# Autodesk Inventor assembly: 1_Base
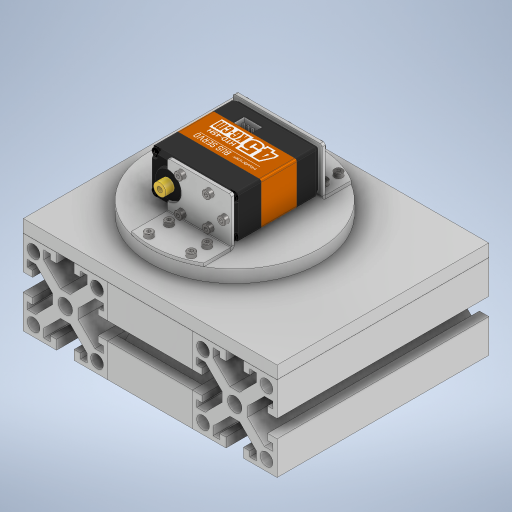
[picture p0: Inventor's stored thumbnail of the model, 512x512]
Saved by Autodesk Inventor 2024.1 (Build 281209000, 209)
## iProperties
Created: 2023-08-24
Part Number: 1_Base
Document SubType Name: Assembly
Designer: chanh
Author: chanh
## Documents named in this file (19)
- C:\Users\chanh\OneDrive - 연세대학교 (Yonsei University)\로봇\Humanoid\Roboin Humanoid Project\Inventor\rh_plus_7_axis_robot_arm_hardware\Assembly\2_Arm.iam
- C:\Users\chanh\OneDrive - 연세대학교 (Yonsei University)\로봇\Humanoid\Roboin Humanoid Project\Inventor\rh_plus_7_axis_robot_arm_hardware\Part\HTD-45H, Horn\HTD-45H\HTD-45H.ipt
- C:\Users\chanh\OneDrive - 연세대학교 (Yonsei University)\로봇\Humanoid\Roboin Humanoid Project\Inventor\rh_plus_7_axis_robot_arm_hardware\Part\Frame\axis_1_top_frame.ipt
- C:\Users\chanh\OneDrive - 연세대학교 (Yonsei University)\로봇\Humanoid\Roboin Humanoid Project\Inventor\rh_plus_7_axis_robot_arm_hardware\Part\Other Parts\Aluminum_Profile_4040_100.14mm_top.ipt
- C:\Users\chanh\OneDrive - 연세대학교 (Yonsei University)\로봇\Humanoid\Roboin Humanoid Project\Inventor\rh_plus_7_axis_robot_arm_hardware\Part\Other Parts\Aluminum_Profile_4040_40.10mm_right.ipt
- C:\Users\chanh\OneDrive - 연세대학교 (Yonsei University)\로봇\Humanoid\Roboin Humanoid Project\Inventor\rh_plus_7_axis_robot_arm_hardware\Part\Other Parts\Aluminum_Profile_4040_40.10mm_left.ipt
- C:\Users\chanh\OneDrive - 연세대학교 (Yonsei University)\로봇\Humanoid\Roboin Humanoid Project\Inventor\rh_plus_7_axis_robot_arm_hardware\Part\Other Parts\Aluminum_Profile_4040_100.14mm_bottom.ipt
- C:\Users\chanh\OneDrive - 연세대학교 (Yonsei University)\로봇\Humanoid\Roboin Humanoid Project\Inventor\rh_plus_7_axis_robot_arm_hardware\Part\HTD-45H, Horn\HTD-45H\M2x32.ipt
- C:\Users\chanh\OneDrive - 연세대학교 (Yonsei University)\로봇\Humanoid\Roboin Humanoid Project\Inventor\rh_plus_7_axis_robot_arm_hardware\Part\HTD-45H, Horn\Horn\Top Horn.ipt
- C:\Users\chanh\OneDrive - 연세대학교 (Yonsei University)\로봇\Humanoid\Roboin Humanoid Project\Inventor\rh_plus_7_axis_robot_arm_hardware\Part\Bolt, Bearing\M2x6 Round Bolt.ipt
- C:\Users\chanh\OneDrive - 연세대학교 (Yonsei University)\로봇\Humanoid\Roboin Humanoid Project\Inventor\rh_plus_7_axis_robot_arm_hardware\Part\Bolt, Bearing\M2x35 Round Bolt.ipt
- C:\Users\chanh\OneDrive - 연세대학교 (Yonsei University)\로봇\Humanoid\Roboin Humanoid Project\Inventor\rh_plus_7_axis_robot_arm_hardware\Part\Frame\axis_2_bottom_frame.ipt
- C:\Users\chanh\OneDrive - 연세대학교 (Yonsei University)\로봇\Humanoid\Roboin Humanoid Project\Inventor\rh_plus_7_axis_robot_arm_hardware\Part\Bolt, Bearing\AXK5070+AS Bearing.ipt
- C:\Users\chanh\OneDrive - 연세대학교 (Yonsei University)\로봇\Humanoid\Roboin Humanoid Project\Inventor\rh_plus_7_axis_robot_arm_hardware\Part\Bolt, Bearing\M2x6 Bolt.ipt
- C:\Users\chanh\OneDrive - 연세대학교 (Yonsei University)\로봇\Humanoid\Roboin Humanoid Project\Inventor\rh_plus_7_axis_robot_arm_hardware\Part\HTD-45H, Horn\HTD-45H\HTD-45H.iam
- C:\Users\chanh\OneDrive - 연세대학교 (Yonsei University)\로봇\Humanoid\Roboin Humanoid Project\Inventor\rh_plus_7_axis_robot_arm_hardware\Part\HTD-45H, Horn\Horn\M3x6.ipt
- C:\Users\chanh\OneDrive - 연세대학교 (Yonsei University)\로봇\Humanoid\Roboin Humanoid Project\Inventor\rh_plus_7_axis_robot_arm_hardware\Part\Frame\axis_2_bottom_L_frame(top).ipt
- C:\Users\chanh\OneDrive - 연세대학교 (Yonsei University)\로봇\Humanoid\Roboin Humanoid Project\Inventor\rh_plus_7_axis_robot_arm_hardware\Part\Frame\axis_2_bottom_L_frame(bottom).ipt
- C:\Users\chanh\OneDrive - 연세대학교 (Yonsei University)\로봇\Humanoid\Roboin Humanoid Project\Inventor\rh_plus_7_axis_robot_arm_hardware\Part\Bolt, Bearing\M2x4 Bolt.ipt
## Components (47 placed, 17 different names)
1. M2x4 Bolt:1 — Rigid:23
2. M2x4 Bolt:2 — Rigid:24
3. M2x4 Bolt:3 — Rigid:25
4. M2x4 Bolt:4 — Rigid:26
5. M2x4 Bolt:5 — Rigid:27
6. M2x4 Bolt:6 — Rigid:28
7. M2x4 Bolt:7 — Rigid:29
8. M2x4 Bolt:8 — Rigid:30
9. M2x4 Bolt:9 — Rigid:31
10. M2x4 Bolt:10 — Rigid:32
11. M2x4 Bolt:11 — Rigid:33
12. M2x4 Bolt:12 — Rigid:34
13. M2x4 Bolt:13 — Rigid:38
14. M2x4 Bolt:14 — Rigid:39
15. M2x4 Bolt:15 — Rigid:41
16. M2x4 Bolt:16 — Rigid:37
17. M2x4 Bolt:17 — Rigid:35
18. M2x4 Bolt:18 — Rigid:36
19. M2x4 Bolt:19 — Rigid:40
20. M2x4 Bolt:20 — Rigid:42
21. M2x4 Bolt:21 — Rigid:43
22. Aluminum_Profile_4040_100.14mm_top:1 — Flush:13, Flush:14, Mate:2, Mate:3, Flush:15, Flush:16, Mate:4, Flush:17, Flush:18, Mate:6
23. Aluminum_Profile_4040_40.10mm_right:1 — Mate:3, Flush:15, Flush:16
24. Aluminum_Profile_4040_40.10mm_left:1 — Mate:4, Flush:17, Flush:18, Mate:5, Flush:20
25. Aluminum_Profile_4040_100.14mm_bottom:1 — Flush:19, Mate:5, Flush:20
26. HTD-45H:1 — Mate:1, Flush:1, Flush:2, Flush:12, Flush:13, Flush:14, Mate:2, Flush:19, Rigid:1, Rigid:2, Rotational:1, Mate:7, Mate:8
27. axis_1_top_frame:1 — Flush:11, Flush:12, Mate:6, Rigid:11, Rigid:12, Rigid:13, Rigid:14, Rigid:15, Rigid:16, Rigid:17, Mate:9
28. HTD-45H:2 [sub-assembly] — Flush:21, Mate:11, Flush:23, Flush:24, Mate:13, Mate:17
29. axis_2_bottom_frame:1 — Rigid:10, Rigid:18, Rigid:19, Rigid:20, Rigid:21, Flush:21, Mate:11, Mate:14
30. axis_2_bottom_L_frame(top):1 — Flush:23, Flush:24, Mate:13, Mate:14, Rigid:23, Rigid:24, Rigid:25, Rigid:26, Rigid:27, Rigid:28, Rigid:29, Rigid:30, Rigid:31
31. axis_2_bottom_L_frame(bottom):1 — Mate:17, Rigid:32, Rigid:33, Rigid:34, Rigid:35, Rigid:36, Rigid:37, Rigid:38, Rigid:39, Rigid:40, Rigid:41, Rigid:42, Rigid:43
32. M2x32:1 — Rigid:2
33. M2x32:2 — Rigid:1
34. Top Horn:1 — Rotational:1, Rigid:10, Rigid:22
35. M3x6:1 — Rigid:22
36. M2x6 Round Bolt:3 — Rigid:16
37. M2x6 Round Bolt:4 — Rigid:17
38. M2x6 Round Bolt:5 — Rigid:15
39. AXK5070+AS Bearing:1 — Mate:7, Mate:8, Mate:9
40. M2x6 Round Bolt:1 — Rigid:14
41. M2x6 Round Bolt:2 — Rigid:13
42. M2x35 Round Bolt:1 — Rigid:11
43. M2x35 Round Bolt:2 — Rigid:12
44. M2x6 Bolt:1 — Rigid:18
45. M2x6 Bolt:2 — Rigid:19
46. M2x6 Bolt:3 — Rigid:20
47. M2x6 Bolt:4 — Rigid:21
## Relationships (65: WeldJoint 36, Flush 15, Mate 13, RevoluteJoint 1)
- Mate:1: HTD-45H:1
- Flush:1: HTD-45H:1
- Flush:2: HTD-45H:1
- Flush:11: axis_1_top_frame:1
- Flush:12: HTD-45H:1 ↔ axis_1_top_frame:1
- Flush:13: Aluminum_Profile_4040_100.14mm_top:1 ↔ HTD-45H:1
- Flush:14: Aluminum_Profile_4040_100.14mm_top:1 ↔ HTD-45H:1
- Mate:2: Aluminum_Profile_4040_100.14mm_top:1 ↔ HTD-45H:1
- Mate:3: Aluminum_Profile_4040_100.14mm_top:1 ↔ Aluminum_Profile_4040_40.10mm_right:1
- Flush:15: Aluminum_Profile_4040_100.14mm_top:1 ↔ Aluminum_Profile_4040_40.10mm_right:1
- Flush:16: Aluminum_Profile_4040_100.14mm_top:1 ↔ Aluminum_Profile_4040_40.10mm_right:1
- Mate:4: Aluminum_Profile_4040_100.14mm_top:1 ↔ Aluminum_Profile_4040_40.10mm_left:1
- Flush:17: Aluminum_Profile_4040_100.14mm_top:1 ↔ Aluminum_Profile_4040_40.10mm_left:1
- Flush:18: Aluminum_Profile_4040_100.14mm_top:1 ↔ Aluminum_Profile_4040_40.10mm_left:1
- Flush:19: Aluminum_Profile_4040_100.14mm_bottom:1 ↔ HTD-45H:1
- Mate:5: Aluminum_Profile_4040_40.10mm_left:1 ↔ Aluminum_Profile_4040_100.14mm_bottom:1
- Flush:20: Aluminum_Profile_4040_40.10mm_left:1 ↔ Aluminum_Profile_4040_100.14mm_bottom:1
- Mate:6: Aluminum_Profile_4040_100.14mm_top:1 ↔ axis_1_top_frame:1
- Rigid:1 [WeldJoint]: HTD-45H:1 ↔ M2x32:2
- Rigid:2 [WeldJoint]: HTD-45H:1 ↔ M2x32:1
- Rotational:1 [RevoluteJoint]: HTD-45H:1 ↔ Top Horn:1
- Rigid:10 [WeldJoint]: axis_2_bottom_frame:1 ↔ Top Horn:1
- Rigid:11 [WeldJoint]: axis_1_top_frame:1 ↔ M2x35 Round Bolt:1
- Rigid:12 [WeldJoint]: axis_1_top_frame:1 ↔ M2x35 Round Bolt:2
- Rigid:13 [WeldJoint]: axis_1_top_frame:1 ↔ M2x6 Round Bolt:2
- Rigid:14 [WeldJoint]: axis_1_top_frame:1 ↔ M2x6 Round Bolt:1
- Rigid:15 [WeldJoint]: axis_1_top_frame:1 ↔ M2x6 Round Bolt:5
- Rigid:16 [WeldJoint]: axis_1_top_frame:1 ↔ M2x6 Round Bolt:3
- Rigid:17 [WeldJoint]: axis_1_top_frame:1 ↔ M2x6 Round Bolt:4
- Mate:7: HTD-45H:1 ↔ AXK5070+AS Bearing:1
- Mate:8: HTD-45H:1 ↔ AXK5070+AS Bearing:1
- Mate:9: axis_1_top_frame:1 ↔ AXK5070+AS Bearing:1
- Rigid:18 [WeldJoint]: axis_2_bottom_frame:1 ↔ M2x6 Bolt:1
- Rigid:19 [WeldJoint]: axis_2_bottom_frame:1 ↔ M2x6 Bolt:2
- Rigid:20 [WeldJoint]: axis_2_bottom_frame:1 ↔ M2x6 Bolt:3
- Rigid:21 [WeldJoint]: axis_2_bottom_frame:1 ↔ M2x6 Bolt:4
- Rigid:22 [WeldJoint]: Top Horn:1 ↔ M3x6:1
- Flush:21: HTD-45H:2 ↔ axis_2_bottom_frame:1
- Mate:11: HTD-45H:2 ↔ axis_2_bottom_frame:1
- Flush:23: HTD-45H:2 ↔ axis_2_bottom_L_frame(top):1
- Flush:24 (-1 mm): HTD-45H:2 ↔ axis_2_bottom_L_frame(top):1
- Mate:13: HTD-45H:2 ↔ axis_2_bottom_L_frame(top):1
- Mate:14: axis_2_bottom_frame:1 ↔ axis_2_bottom_L_frame(top):1
- Mate:17: HTD-45H:2 ↔ axis_2_bottom_L_frame(bottom):1
- Rigid:23 [WeldJoint]: M2x4 Bolt:1 ↔ axis_2_bottom_L_frame(top):1
- Rigid:24 [WeldJoint]: M2x4 Bolt:2 ↔ axis_2_bottom_L_frame(top):1
- Rigid:25 [WeldJoint]: M2x4 Bolt:3 ↔ axis_2_bottom_L_frame(top):1
- Rigid:26 [WeldJoint]: M2x4 Bolt:4 ↔ axis_2_bottom_L_frame(top):1
- Rigid:27 [WeldJoint]: M2x4 Bolt:5 ↔ axis_2_bottom_L_frame(top):1
- Rigid:28 [WeldJoint]: M2x4 Bolt:6 ↔ axis_2_bottom_L_frame(top):1
- Rigid:29 [WeldJoint]: M2x4 Bolt:7 ↔ axis_2_bottom_L_frame(top):1
- Rigid:30 [WeldJoint]: M2x4 Bolt:8 ↔ axis_2_bottom_L_frame(top):1
- Rigid:31 [WeldJoint]: M2x4 Bolt:9 ↔ axis_2_bottom_L_frame(top):1
- Rigid:32 [WeldJoint]: M2x4 Bolt:10 ↔ axis_2_bottom_L_frame(bottom):1
- Rigid:33 [WeldJoint]: M2x4 Bolt:11 ↔ axis_2_bottom_L_frame(bottom):1
- Rigid:34 [WeldJoint]: M2x4 Bolt:12 ↔ axis_2_bottom_L_frame(bottom):1
- Rigid:35 [WeldJoint]: M2x4 Bolt:17 ↔ axis_2_bottom_L_frame(bottom):1
- Rigid:36 [WeldJoint]: M2x4 Bolt:18 ↔ axis_2_bottom_L_frame(bottom):1
- Rigid:37 [WeldJoint]: M2x4 Bolt:16 ↔ axis_2_bottom_L_frame(bottom):1
- Rigid:38 [WeldJoint]: M2x4 Bolt:13 ↔ axis_2_bottom_L_frame(bottom):1
- Rigid:39 [WeldJoint]: M2x4 Bolt:14 ↔ axis_2_bottom_L_frame(bottom):1
- Rigid:40 [WeldJoint]: M2x4 Bolt:19 ↔ axis_2_bottom_L_frame(bottom):1
- Rigid:41 [WeldJoint]: M2x4 Bolt:15 ↔ axis_2_bottom_L_frame(bottom):1
- Rigid:42 [WeldJoint]: M2x4 Bolt:20 ↔ axis_2_bottom_L_frame(bottom):1
- Rigid:43 [WeldJoint]: M2x4 Bolt:21 ↔ axis_2_bottom_L_frame(bottom):1
